# Autodesk Inventor assembly: MS5607
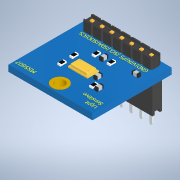
[picture p0: Inventor's stored thumbnail of the model, 180x180]
Saved by Autodesk Inventor 2022 (Build 260153000, 153)
## iProperties
Created: 2022-03-16
Part Number: MS5607
Document SubType Name: Assembly
Designer: dvorakj
Author: dvorakj
## Documents named in this file (7)
- C:\Users\dvorakj\Documents\Inventor\Bakalarka\MS5607\MS5607.iam
- C:\Users\dvorakj\Documents\Inventor\Bakalarka\MS5607\MS5607_pcb.ipt
- C:\Users\dvorakj\Documents\Inventor\Bakalarka\MS5607\Senzor\User Library-MS5607-02BA03.iam
- C:\Users\dvorakj\Documents\Inventor\Bakalarka\MS5607\Pin header\61300711121 (rev1)plastic on top.iam
- C:\Users\dvorakj\Documents\Inventor\Bakalarka\Common\CAP\Download_STP_8850122060xx (rev1).iam
- C:\Users\dvorakj\Documents\Inventor\Bakalarka\Common\RES\Resistor_0603.iam
- C:\Users\dvorakj\Documents\Inventor\Bakalarka\Common\Header7p\header7p.iam
## Components (13 placed, 6 different names)
1. MS5607_pcb:1 — Mate:2, Angle:1, Mate:3, Mate:4, Flush:9, Mate:6
2. User Library-MS5607-02BA03:1 [sub-assembly] — Mate:2, Angle:1, Flush:9
3. 61300711121 (rev1)plastic on top:1 [sub-assembly] — Mate:3, Mate:5, Angle:2
4. Download_STP_8850122060xx (rev1):1 [sub-assembly] — Flush:2, Flush:3
5. Download_STP_8850122060xx (rev1):2 [sub-assembly] — Flush:3, Flush:4, Flush:5
6. Download_STP_8850122060xx (rev1):3 [sub-assembly] — Flush:1, Flush:2, Mate:4
7. Resistor_0603:1 [sub-assembly] — Flush:5
8. Resistor_0603:2 [sub-assembly] — Flush:7, Flush:8
9. Resistor_0603:3 [sub-assembly] — Flush:8
10. Resistor_0603:4 [sub-assembly] — Flush:4, Flush:6
11. Resistor_0603:5 [sub-assembly] — Flush:6, Flush:7
12. Download_STP_8850122060xx (rev1):4 [sub-assembly] — Flush:1
13. header7p:1 [sub-assembly] — Mate:5, Angle:2, Mate:6
## Relationships (16: Flush 9, Mate 5, Angle 2)
- Mate:2: MS5607_pcb:1 ↔ User Library-MS5607-02BA03:1
- Angle:1 (0 deg): MS5607_pcb:1 ↔ User Library-MS5607-02BA03:1
- Mate:3: MS5607_pcb:1 ↔ 61300711121 (rev1)plastic on top:1
- Flush:1: Download_STP_8850122060xx (rev1):3 ↔ Download_STP_8850122060xx (rev1):4
- Flush:2: Download_STP_8850122060xx (rev1):1 ↔ Download_STP_8850122060xx (rev1):3
- Flush:3: Download_STP_8850122060xx (rev1):1 ↔ Download_STP_8850122060xx (rev1):2
- Flush:4: Download_STP_8850122060xx (rev1):2 ↔ Resistor_0603:4
- Flush:5: Download_STP_8850122060xx (rev1):2 ↔ Resistor_0603:1
- Flush:6: Resistor_0603:4 ↔ Resistor_0603:5
- Flush:7: Resistor_0603:2 ↔ Resistor_0603:5
- Flush:8: Resistor_0603:2 ↔ Resistor_0603:3
- Mate:4: MS5607_pcb:1 ↔ Download_STP_8850122060xx (rev1):3
- Flush:9 (7 mm): MS5607_pcb:1 ↔ User Library-MS5607-02BA03:1
- Mate:5: 61300711121 (rev1)plastic on top:1 ↔ header7p:1
- Angle:2 (0 deg): 61300711121 (rev1)plastic on top:1 ↔ header7p:1
- Mate:6: MS5607_pcb:1 ↔ header7p:1
